# Autodesk Inventor assembly: 0hnks
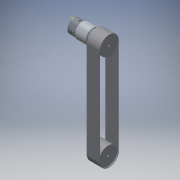
[picture p0: Inventor's stored thumbnail of the model, 180x180]
Saved by Autodesk Inventor 2019 (Build 230136000, 136)
## iProperties
Created: 2021-12-23
Part Number: 0hnks
Material: 一般
Document SubType Name: Assembly
Designer: yuta
Author: yuta
## Documents named in this file (4)
- C:\Users\yuta\Documents\キャチロボ\0hnks.iam
- C:\Users\yuta\Documents\キャチロボ\0nhk.ipt
- C:\Users\yuta\Documents\キャチロボ\0nhk2.ipt
- C:\Users\yuta\Documents\キャチロボ\RS775_CAD_IAM\モーター RS775-8513DF.iam
## Components (4 placed, 3 different names)
1. 0nhk:1 — メイト:1, メイト:2
2. 0nhk2:1 — メイト:1, メイト:3
3. モーター RS775-8513DF:2 [sub-assembly] — メイト:3
4. 0nhk2:2 — メイト:2
## Relationships (3: Mate 3)
- メイト:1 [Mate]: 0nhk:1 ↔ 0nhk2:1
- メイト:2 [Mate]: 0nhk:1 ↔ 0nhk2:2
- メイト:3 [Mate]: 0nhk2:1 ↔ モーター RS775-8513DF:2
